# Autodesk Inventor assembly: Drive Wheel Assembly with Perf Wheels
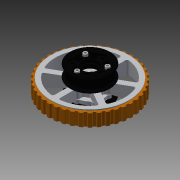
[picture p0: Inventor's stored thumbnail of the model, 180x180]
Saved by Autodesk Inventor 2013 (Build 170138000, 138)
## iProperties
Created: 2013-02-07
Part Number: Drive Wheel Assembly with Perf Wheels
Document SubType Name: Assembly
Designer: Moses
Author: Moses
## Documents named in this file (5)
- C:\Users\Moses\Documents\GitHub\frc2013CAD\Drivetrain\Drive Wheel Assembly with Perf Wheels.iam
- C:\Users\Moses\Documents\GitHub\frc2013CAD\Drivetrain\6 Perf ThruTread 500 Hex\6 Perf Plaction Tread 500 Hex.iam
- C:\Users\Moses\Documents\GitHub\frc2013CAD\Drivetrain\DBK_42ToothPulley (am-2234)\DBK_42ToothPulley V2.iam
- C:\Users\Moses\Documents\GitHub\frc2013CAD\Drivetrain\Custom Belt Pulley Hex Hub.ipt
- C:\Users\Moses\Documents\GitHub\frc2013CAD\Drivetrain\91251A980 10-24 Screw\91251A980.ipt
## Components (8 placed, 4 different names)
1. 6 Perf Plaction Tread 500 Hex:1 [sub-assembly] — Mate:7, Mate:8, Mate:9, Tangent:1, Mate:10, Mate:11
2. DBK_42ToothPulley V2:1 [sub-assembly] — Tangent:1, Mate:10, Mate:11, Insert:1, Insert:2, Insert:3
3. DBK_42ToothPulley V2:2 [sub-assembly] — Mate:1, Mate:2, Mate:3, Mate:8, Mate:9
4. Custom Belt Pulley Hex Hub:1 — Mate:1, Mate:2, Mate:3, Mate:4, Mate:5, Mate:6
5. Custom Belt Pulley Hex Hub:2 — Mate:4, Mate:5, Mate:6, Mate:7
6. 91251A980:1 — Insert:2
7. 91251A980:2 — Insert:3
8. 91251A980:3 — Insert:1
## Relationships (15: Mate 11, Insert 3, Tangent 1)
- Mate:1: DBK_42ToothPulley V2:2 ↔ Custom Belt Pulley Hex Hub:1
- Mate:2: DBK_42ToothPulley V2:2 ↔ Custom Belt Pulley Hex Hub:1
- Mate:3: DBK_42ToothPulley V2:2 ↔ Custom Belt Pulley Hex Hub:1
- Mate:4: Custom Belt Pulley Hex Hub:1 ↔ Custom Belt Pulley Hex Hub:2
- Mate:5: Custom Belt Pulley Hex Hub:1 ↔ Custom Belt Pulley Hex Hub:2
- Mate:6: Custom Belt Pulley Hex Hub:1 ↔ Custom Belt Pulley Hex Hub:2
- Mate:7: 6 Perf Plaction Tread 500 Hex:1 ↔ Custom Belt Pulley Hex Hub:2
- Mate:8: 6 Perf Plaction Tread 500 Hex:1 ↔ DBK_42ToothPulley V2:2
- Mate:9: 6 Perf Plaction Tread 500 Hex:1 ↔ DBK_42ToothPulley V2:2
- Tangent:1: 6 Perf Plaction Tread 500 Hex:1 ↔ DBK_42ToothPulley V2:1
- Mate:10: 6 Perf Plaction Tread 500 Hex:1 ↔ DBK_42ToothPulley V2:1
- Mate:11: 6 Perf Plaction Tread 500 Hex:1 ↔ DBK_42ToothPulley V2:1
- Insert:1: DBK_42ToothPulley V2:1 ↔ 91251A980:3
- Insert:2: DBK_42ToothPulley V2:1 ↔ 91251A980:1
- Insert:3: DBK_42ToothPulley V2:1 ↔ 91251A980:2
